# Autodesk Inventor assembly: HS 48T Gear, No Insert, Lathe_MIR_MIR
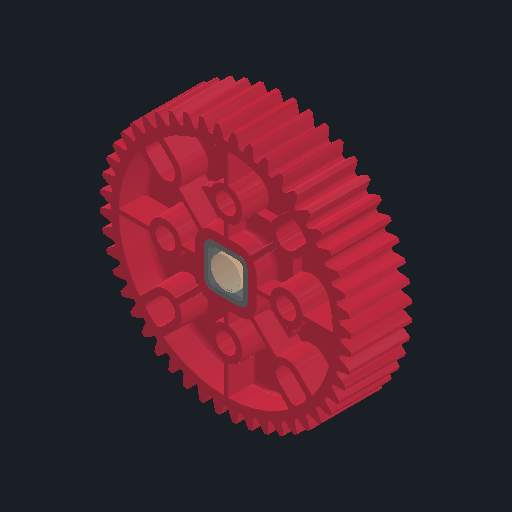
[picture p0: Inventor's stored thumbnail of the model, 512x512]
Saved by Autodesk Inventor 2026.1 (Build 301233000, 233)
## iProperties
Created: 2022-08-02
Part Number: HS 48T Gear, No Insert, Lathe_MIR_MIR
Document SubType Name: Assembly
Designer: roejo
Author: ylu12
## Documents named in this file (2)
- C:\Users\roejo\OneDrive\Documents\2026WorldChampionRobot\Library\Custom Parts\HS 48T Gear, No Insert, Lathe_MIR_MIR.iam
- C:\Users\roejo\OneDrive\Documents\2026WorldChampionRobot\Library\VEX-CAD-Inventor-1.4.2\Motion\Gears\Reference Files\HS 48T Gear, No Insert_MIR_MIR.ipt
## Components (1 placed, 1 different names)
1. HS 48T Gear, No Insert_MIR_MIR:1 — Flush:6, Mate:11, Mate:12
## Relationships (3: Mate 2, Flush 1)
- Flush:6: HS 48T Gear, No Insert_MIR_MIR:1
- Mate:11: HS 48T Gear, No Insert_MIR_MIR:1
- Mate:12: HS 48T Gear, No Insert_MIR_MIR:1
